# Autodesk Inventor assembly: Assem
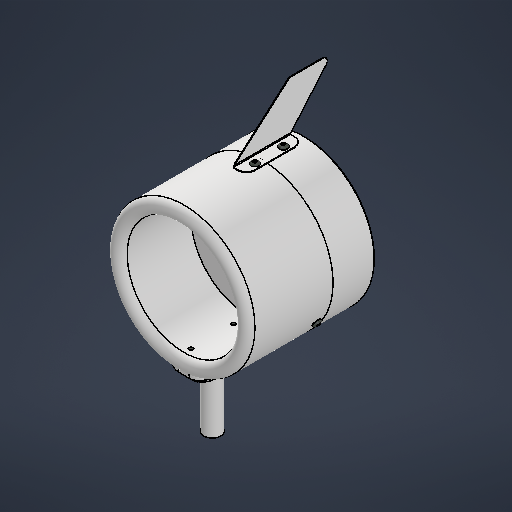
[picture p0: Inventor's stored thumbnail of the model, 512x512]
Saved by Autodesk Inventor 2026.1 (Build 301233000, 233)
## iProperties
Created: 2025-09-27
Part Number: Assem
Document SubType Name: Assembly
Designer: 1char
Mass: 239.26 g
Surface Area: 868.338 cm^2
Volume: 234.532 cm^3
Density: 1.02016 g/cm^3
Author: 1char
## Documents named in this file (8)
- C:\Users\1char\Documents\Plastic_Duct\Assem.iam
- C:\Users\1char\Documents\Plastic_Duct\Filter.ipt
- C:\Users\1char\Documents\Plastic_Duct\Nose.ipt
- C:\Users\1char\Documents\Plastic_Duct\Tail.ipt
- C:\Users\1char\Documents\Inventor\Content Center Files\R2026\en-US\ISO 7380-1\ISO 7380-1 - M3 x 10.ipt
- C:\Users\1char\Documents\Plastic_Duct\Mount_A.ipt
- C:\Users\1char\Documents\Plastic_Duct\Fin.ipt
- C:\Users\1char\Documents\Inventor\Content Center Files\R2026\en-US\ISO 7380-1\ISO 7380-1 - M3 x 16.ipt
## Components (11 placed, 7 different names)
1. Filter:1 — Mate:1, Mate:7
2. Nose:1 — Mate:1, Mate:2, Rigid:1, Mate:3, Mate:4, Mate:6, Mate:7
3. Tail:1 — Mate:2, Mate:5, Mate:6, Tangent:1
4. Mount_A:1 — Mate:3, Mate:4, Rigid:2, Rigid:3
5. Fin:1 — Mate:5, Mate:8, Tangent:1, Rotational:1, Angle:1
6. ISO 7380-1 M3 x 10:4 — Rotational:1
7. ISO 7380-1 M3 x 16:1 — Rigid:2
8. ISO 7380-1 M3 x 16:2 — Rigid:3
9. ISO 7380-1 M3 x 10:1 — Rigid:1, Mate:8
10. ISO 7380-1 M3 x 10:2
11. ISO 7380-1 M3 x 10:3
## Component patterns: (3 elements, first: ISO 7380-1 M3 x 10:1)
## Relationships (14: Mate 8, WeldJoint 3, Tangent 1, RevoluteJoint 1, Angle 1)
- Mate:1: Filter:1 ↔ Nose:1
- Mate:2: Nose:1 ↔ Tail:1
- Rigid:1 [WeldJoint]: Nose:1 ↔ ISO 7380-1 M3 x 10:1
- Mate:3: Nose:1 ↔ Mount_A:1
- Mate:4: Nose:1 ↔ Mount_A:1
- Mate:5: Tail:1 ↔ Fin:1
- Mate:6: Nose:1 ↔ Tail:1
- Mate:7: Filter:1 ↔ Nose:1
- Mate:8: Fin:1 ↔ ISO 7380-1 M3 x 10:1
- Tangent:1: Tail:1 ↔ Fin:1
- Rotational:1 [RevoluteJoint]: Fin:1 ↔ ISO 7380-1 M3 x 10:4
- Angle:1 (0 deg): Fin:1
- Rigid:2 [WeldJoint]: Mount_A:1 ↔ ISO 7380-1 M3 x 16:1
- Rigid:3 [WeldJoint]: Mount_A:1 ↔ ISO 7380-1 M3 x 16:2
